# Autodesk Inventor assembly: Talon with Fan
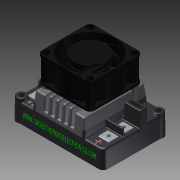
[picture p0: Inventor's stored thumbnail of the model, 180x180]
Saved by Autodesk Inventor 2013 (Build 170138000, 138)
## iProperties
Created: 2013-01-27
Part Number: Talon with Fan
Document SubType Name: Assembly
Designer: Moses
Mass: 102.554 g
Surface Area: 523.107 cm^2
Volume: 54.4985 cm^3
Density: 1.88178 g/cm^3
Author: Moses
## Documents named in this file (3)
- C:\Users\Moses\Documents\GitHub\frc2013CAD\Electrical\Talon with Fan.iam
- C:\Users\Moses\Documents\GitHub\frc2013CAD\Electrical\Talon.ipt
- C:\Users\Moses\Documents\GitHub\frc2013CAD\Electrical\ELEC_FanMini_412.iam
## Components (2 placed, 2 different names)
1. Talon:1 — Mate:1, Mate:2, Mate:3
2. ELEC_FanMini_412:1 [sub-assembly] — Mate:1, Mate:2, Mate:3
## Relationships (3: Mate 3)
- Mate:1: Talon:1 ↔ ELEC_FanMini_412:1
- Mate:2 (14.4018 mm): Talon:1 ↔ ELEC_FanMini_412:1
- Mate:3 (4.2418 mm): Talon:1 ↔ ELEC_FanMini_412:1
